# Autodesk Inventor assembly: McCrea_head_walle
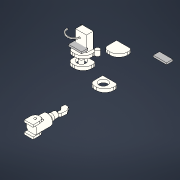
[picture p0: Inventor's stored thumbnail of the model, 180x180]
Saved by Autodesk Inventor 2022 (Build 260153000, 153)
## iProperties
Created: 2022-01-20
Part Number: McCrea_head_walle
Document SubType Name: Assembly
Designer: MatusBarany
Author: MatusBarany
## Documents named in this file (12)
- C:\Users\MatusBarany\Documents\Inventor\wall-e\assembly\McCrea_head_walle.iam
- C:\Users\MatusBarany\Documents\Inventor\wall-e\maxo\McCrea_kabel_walle.ipt
- C:\Users\MatusBarany\Documents\Inventor\wall-e\maxo\McCrea_krk_walle.ipt
- C:\Users\MatusBarany\Documents\Inventor\wall-e\maxo\McCrea_oblucik_walle.ipt
- C:\Users\MatusBarany\Documents\Inventor\wall-e\maxo\McCrea_oko_walle.ipt
- C:\Users\MatusBarany\Documents\Inventor\wall-e\maxo\McCrea_palicka_walle.ipt
- C:\Users\MatusBarany\Documents\Inventor\wall-e\maxo\McCrea_uhco_walle.ipt
- C:\Users\MatusBarany\Documents\Inventor\wall-e\maxo\McCrea_velka_palicka_walle.ipt
- C:\Users\MatusBarany\Documents\Inventor\wall-e\maxo\McCrea_velka_palicka_walle_1.ipt
- C:\Users\MatusBarany\Documents\Inventor\wall-e\maxo\McCrea_velky_krk_walle.ipt
- C:\Users\MatusBarany\Documents\Inventor\wall-e\maxo\McCrea_zadna_cast_oka_walle.ipt
- C:\Users\MatusBarany\Documents\Inventor\wall-e\maxo\McCrea_zadne_oko_walle.ipt
## Components (16 placed, 11 different names)
1. McCrea_krk_walle:1 — Rigid:1, Rigid:2
2. McCrea_oblucik_walle:1 — Rotational:2, Rigid:2
3. McCrea_oko_walle:1
4. McCrea_palicka_walle:1 — Rotational:1
5. McCrea_uhco_walle:1
6. McCrea_zadna_cast_oka_walle:1
7. McCrea_kabel_walle:2
8. McCrea_oblucik_walle:2 — Rotational:1, Rigid:1
9. McCrea_oko_walle:2
10. McCrea_palicka_walle:2 — Rotational:2
11. McCrea_uhco_walle:2
12. McCrea_velka_palicka_walle:2
13. McCrea_velka_palicka_walle_1:2
14. McCrea_velky_krk_walle:2
15. McCrea_zadna_cast_oka_walle:2
16. McCrea_zadne_oko_walle:2
## Relationships (4: RevoluteJoint 2, WeldJoint 2)
- Rotational:1 [RevoluteJoint]: McCrea_palicka_walle:1 ↔ McCrea_oblucik_walle:2
- Rigid:1 [WeldJoint]: McCrea_krk_walle:1 ↔ McCrea_oblucik_walle:2
- Rotational:2 [RevoluteJoint]: McCrea_oblucik_walle:1 ↔ McCrea_palicka_walle:2
- Rigid:2 [WeldJoint]: McCrea_krk_walle:1 ↔ McCrea_oblucik_walle:1
